# Autodesk Inventor assembly: drivenAFrame
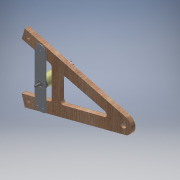
[picture p0: Inventor's stored thumbnail of the model, 180x180]
Saved by Autodesk Inventor 2018 (Build 220112000, 112)
## iProperties
Created: 2017-05-09
Part Number: drivenAFrame
Document SubType Name: Assembly
Designer: admin
Author: admin
## Documents named in this file (5)
- C:\Users\admin\Desktop\RoboEaglesCad2018\drivenAFrame.iam
- C:\Users\admin\Desktop\RoboEaglesCad2018\aFrameBase.ipt
- C:\Users\admin\Desktop\RoboEaglesCad2018\RoboEagles2017\PG188withMotor.ipt
- C:\Users\admin\Desktop\RoboEaglesCad2018\FR8ZZ Hex Bearing.ipt
- C:\Users\admin\Desktop\RoboEaglesCad2018\newPG188Mount.ipt
## Components (4 placed, 4 different names)
1. aFrameBase:1 — Insert:2, Mate:1, Mate:2, Mate:3
2. PG188withMotor:1 — Insert:3, Insert:4, Insert:5
3. FR8ZZ Hex Bearing:1 — Insert:2
4. newPG188Mount:1 — Insert:3, Insert:4, Insert:5, Mate:1, Mate:2, Mate:3
## Relationships (7: Insert 4, Mate 3)
- Insert:2: aFrameBase:1 ↔ FR8ZZ Hex Bearing:1
- Insert:3: PG188withMotor:1 ↔ newPG188Mount:1
- Insert:4: PG188withMotor:1 ↔ newPG188Mount:1
- Insert:5: PG188withMotor:1 ↔ newPG188Mount:1
- Mate:1: aFrameBase:1 ↔ newPG188Mount:1
- Mate:2: aFrameBase:1 ↔ newPG188Mount:1
- Mate:3: aFrameBase:1 ↔ newPG188Mount:1
